# Autodesk Inventor assembly: Assembly1
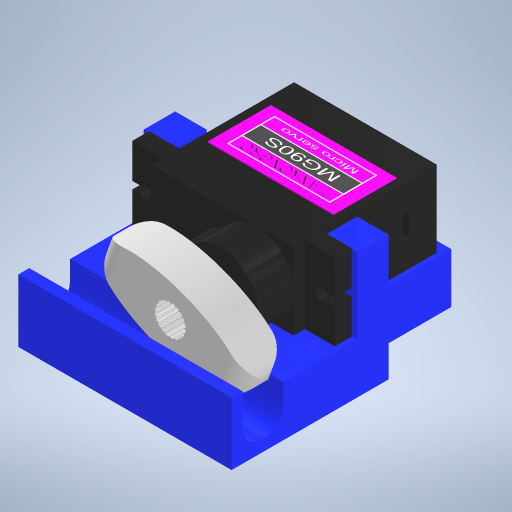
[picture p0: Inventor's stored thumbnail of the model, 512x512]
Saved by Autodesk Inventor 2024.4 (Build 284460000, 460)
## iProperties
Created: 2026-06-02
Part Number: Assembly1
Document SubType Name: Assembly
Designer: Apleppli
Author: Apleppli
## Documents named in this file (4)
- D:\Downloads\Base_servo\Assembly1.iam
- D:\Downloads\Base_servo\base.ipt
- D:\Downloads\Base_servo\MG90S\ServoMG90S.iam
- D:\Downloads\Base_servo\bloqueadorXD.ipt
## Components (3 placed, 3 different names)
1. base:1 — Mate:4, Mate:7, Mate:8, Mate:9
2. ServoMG90S:1 [sub-assembly] — Mate:4, Mate:6, Mate:8, Mate:9
3. bloqueadorXD:1 — Mate:6, Mate:7
## Relationships (5: Mate 5)
- Mate:4: base:1 ↔ ServoMG90S:1
- Mate:6: ServoMG90S:1 ↔ bloqueadorXD:1
- Mate:7: base:1 ↔ bloqueadorXD:1
- Mate:8 (0.65 mm): base:1 ↔ ServoMG90S:1
- Mate:9: base:1 ↔ ServoMG90S:1
